# Autodesk Inventor assembly: cafetiera
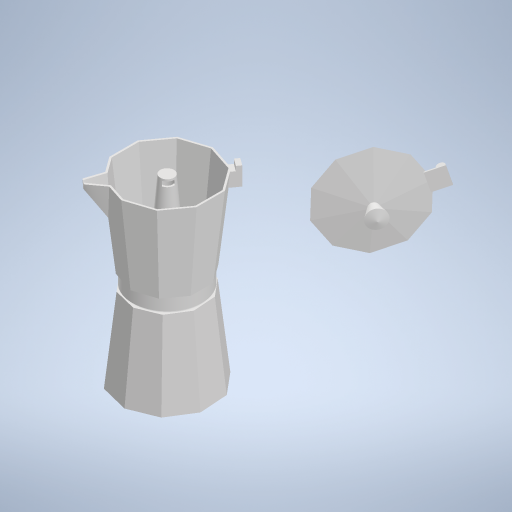
[picture p0: Inventor's stored thumbnail of the model, 512x512]
Saved by Autodesk Inventor 2024 (Build 280153000, 153)
## iProperties
Created: 2024-01-16
Part Number: cafetiera
Document SubType Name: Assembly
Designer: Sorin
Author: Sorin
## Documents named in this file (6)
- C:\Users\Sorin\modelare 3D\cafetiera.iam
- C:\Users\Sorin\modelare 3D\corp.ipt
- C:\Users\Sorin\modelare 3D\capac.ipt
- C:\Users\Sorin\modelare 3D\comp.ipt
- C:\Users\Sorin\modelare 3D\partea_de_jos.ipt
- C:\Users\Sorin\modelare 3D\sita.ipt
## Components (5 placed, 5 different names)
1. corp:1 — Rotational:1, Rotational:2, Angle:1
2. capac:1 — Angle:1, Rotational:3
3. comp:1 — Rotational:3
4. partea_de_jos:1 — Rotational:2
5. sita:1 — Rotational:1
## Relationships (4: RevoluteJoint 3, Angle 1)
- Rotational:1 [RevoluteJoint]: corp:1 ↔ sita:1
- Rotational:2 [RevoluteJoint]: corp:1 ↔ partea_de_jos:1
- Angle:1 (0 deg): corp:1 ↔ capac:1
- Rotational:3 [RevoluteJoint]: capac:1 ↔ comp:1
